# Autodesk Inventor assembly: SpiritBot V1.0
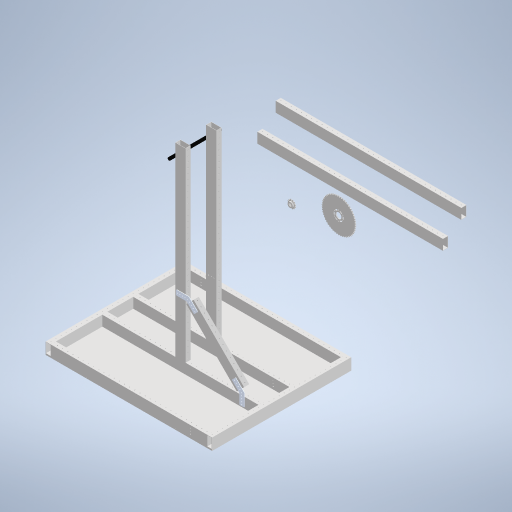
[picture p0: Inventor's stored thumbnail of the model, 512x512]
Saved by Autodesk Inventor 2024 (Build 280153000, 153)
## iProperties
Created: 2023-07-06
Part Number: SpiritBot V1.0
Document SubType Name: Assembly
Designer: Gabriel Marquez
Author: Gabriel Marquez
## Documents named in this file (11)
- C:\Users\Gabriel Marquez\OneDrive\Documents\GitHub\T3-CAD\Current Season CAD\SpiritBot V1.0.iam
- C:\Users\Gabriel Marquez\OneDrive\Documents\GitHub\T3-CAD\Current Season CAD\Body\Base.ipt
- C:\Users\Gabriel Marquez\OneDrive\Documents\GitHub\T3-CAD\Current Season CAD\Body\Long bar 3- VersaFrame.ipt
- C:\Users\Gabriel Marquez\OneDrive\Documents\GitHub\T3-CAD\Current Season CAD\Body\Long bar 4- VersaFrame.ipt
- C:\Users\Gabriel Marquez\OneDrive\Documents\GitHub\T3-CAD\Current Season CAD\Body\Long bar 8.5 - VersaFrame.ipt
- C:\Users\Gabriel Marquez\OneDrive\Documents\GitHub\T3-CAD\Current Season CAD\Body\Long bar 32.3 - VersaFrame.ipt
- C:\Users\Gabriel Marquez\OneDrive\Documents\GitHub\T3-CAD\Stock\Versa System\Gussets\135 Degree Gusset.ipt
- C:\Users\Gabriel Marquez\OneDrive\Documents\GitHub\T3-CAD\Current Season CAD\Body\Super Structure ThunderHex.ipt
- C:\Users\Gabriel Marquez\OneDrive\Documents\GitHub\T3-CAD\Stock\Belts-Chain\Chain\#35\Sprockets\12 Tooth Single.ipt
- C:\Users\Gabriel Marquez\OneDrive\Documents\GitHub\T3-CAD\Stock\Belts-Chain\Chain\#35\Sprockets\54 Tooth plate sprocket.ipt
- C:\Users\Gabriel Marquez\OneDrive\Documents\GitHub\T3-CAD\Current Season CAD\Body\gun turret main spar.ipt
## Components (17 placed, 10 different names)
1. Base:1 — Mate:7, Mate:8
2. Long bar 32.3 - VersaFrame:1 — Mate:1, Mate:2, Mate:6, Mate:7, Mate:14
3. Long bar 32.3 - VersaFrame:2 — Mate:5, Mate:26
4. Long bar 32.3 - VersaFrame:3 — Mate:10, Mate:11, Mate:14, Mate:15, Mate:16, Rotational:1, Rotational:2
5. Long bar 8.5 - VersaFrame:1 — Mate:1, Mate:2, Mate:5, Mate:11, Mate:24
6. Long bar 8.5 - VersaFrame:2 — Mate:6, Mate:8, Mate:10, Mate:20, Mate:23
7. Long bar 3- VersaFrame:2 — Mate:15, Mate:16, Mate:20, Mate:25, Rotational:4, Rotational:5
8. Long bar 32.3 - VersaFrame:4 — Mate:23, Mate:24, Mate:26
9. Long bar 3- VersaFrame:3 — Mate:25
10. 135 Degree Gusset:11 — Rotational:1, Rotational:2, Rotational:3
11. Long bar 4- VersaFrame:1 — Rotational:3
12. 135 Degree Gusset:12 — Rotational:4, Rotational:5
13. Super Structure ThunderHex:1
14. 12 Tooth Single:1
15. 54 Tooth plate sprocket:1
16. gun turret main spar:1
17. gun turret main spar:2
## Relationships (25: Mate 20, RevoluteJoint 5)
- Mate:1: Long bar 32.3 - VersaFrame:1 ↔ Long bar 8.5 - VersaFrame:1
- Mate:2: Long bar 32.3 - VersaFrame:1 ↔ Long bar 8.5 - VersaFrame:1
- [Mate]: Long bar 32.3 - VersaFrame:2 ↔ Long bar 8.5 - VersaFrame:2
- [Mate]: Long bar 32.3 - VersaFrame:2 ↔ Long bar 8.5 - VersaFrame:2
- Mate:5: Long bar 32.3 - VersaFrame:2 ↔ Long bar 8.5 - VersaFrame:1
- Mate:6: Long bar 32.3 - VersaFrame:1 ↔ Long bar 8.5 - VersaFrame:2
- Mate:7: Base:1 ↔ Long bar 32.3 - VersaFrame:1
- Mate:8: Base:1 ↔ Long bar 8.5 - VersaFrame:2
- Mate:10: Long bar 32.3 - VersaFrame:3 ↔ Long bar 8.5 - VersaFrame:2
- Mate:11: Long bar 32.3 - VersaFrame:3 ↔ Long bar 8.5 - VersaFrame:1
- Mate:14 (228.6 mm): Long bar 32.3 - VersaFrame:1 ↔ Long bar 32.3 - VersaFrame:3
- Mate:15: Long bar 32.3 - VersaFrame:3 ↔ Long bar 3- VersaFrame:2
- Mate:16: Long bar 32.3 - VersaFrame:3 ↔ Long bar 3- VersaFrame:2
- Mate:20 (359.41 mm): Long bar 8.5 - VersaFrame:2 ↔ Long bar 3- VersaFrame:2
- [Mate]: Long bar 32.3 - VersaFrame:4 ↔ Long bar 3- VersaFrame:3
- [Mate]: Long bar 32.3 - VersaFrame:4 ↔ Long bar 3- VersaFrame:3
- Mate:23: Long bar 8.5 - VersaFrame:2 ↔ Long bar 32.3 - VersaFrame:4
- Mate:24: Long bar 8.5 - VersaFrame:1 ↔ Long bar 32.3 - VersaFrame:4
- Mate:25: Long bar 3- VersaFrame:2 ↔ Long bar 3- VersaFrame:3
- Mate:26 (228.6 mm): Long bar 32.3 - VersaFrame:2 ↔ Long bar 32.3 - VersaFrame:4
- Rotational:1 [RevoluteJoint]: Long bar 32.3 - VersaFrame:3 ↔ 135 Degree Gusset:11
- Rotational:2 [RevoluteJoint]: Long bar 32.3 - VersaFrame:3 ↔ 135 Degree Gusset:11
- Rotational:3 [RevoluteJoint]: 135 Degree Gusset:11 ↔ Long bar 4- VersaFrame:1
- Rotational:4 [RevoluteJoint]: Long bar 3- VersaFrame:2 ↔ 135 Degree Gusset:12
- Rotational:5 [RevoluteJoint]: Long bar 3- VersaFrame:2 ↔ 135 Degree Gusset:12
## Named parameters: d2_d0 = 0 mm, d3_d1 = 0 mm, d62_d14 = 0 mm, d63_d15 = 0 mm
